# Autodesk Inventor assembly: for_bool
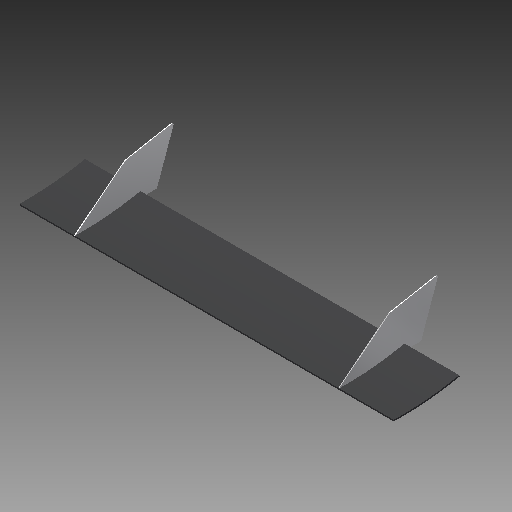
[picture p0: Inventor's stored thumbnail of the model, 512x512]
Saved by Autodesk Inventor 2018 (Build 220112000, 112)
## iProperties
Created: 2017-10-25
Part Number: for_bool
Material: 一般
Document SubType Name: Assembly
Designer: kuwano
Author: kuwano
## Documents named in this file (3)
- Z:\個人フォルダ\kuwano\Inventor\KS-15_Aero_CAD\type5\F-wing\parts\base\for_bool.iam
- Z:\個人フォルダ\kuwano\Inventor\KS-15_Aero_CAD\type5\F-wing\parts\base\base.ipt
- Z:\個人フォルダ\kuwano\Inventor\KS-15_Aero_CAD\type5\F-wing\parts\stay_middle.ipt
## Components (3 placed, 2 different names)
1. base:1 — フラッシュ:1, フラッシュ:2, フラッシュ:3, メイト:1, メイト:2, メイト:3, メイト:4, フラッシュ:4, フラッシュ:5
2. stay_middle:1 — メイト:1, メイト:3, フラッシュ:5
3. stay_middle:2 — メイト:2, メイト:4, フラッシュ:4
## Relationships (9: Flush 5, Mate 4)
- フラッシュ:1 [Flush]: base:1
- フラッシュ:2 [Flush]: base:1
- フラッシュ:3 [Flush]: base:1
- メイト:1 [Mate]: base:1 ↔ stay_middle:1
- メイト:2 [Mate]: base:1 ↔ stay_middle:2
- メイト:3 [Mate]: base:1 ↔ stay_middle:1
- メイト:4 [Mate]: base:1 ↔ stay_middle:2
- フラッシュ:4 [Flush] (200 mm): base:1 ↔ stay_middle:2
- フラッシュ:5 [Flush] (200 mm): base:1 ↔ stay_middle:1
